# Autodesk Inventor assembly: belt drives
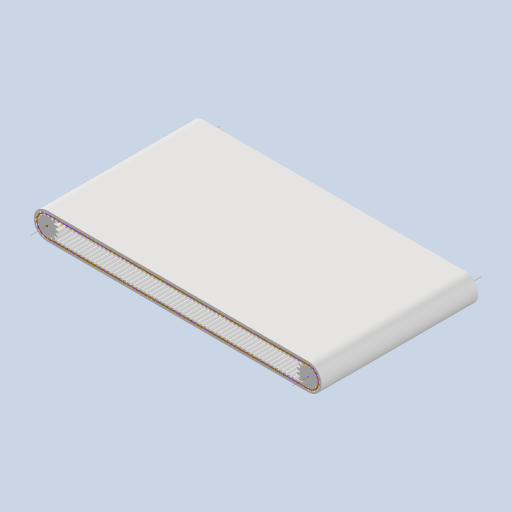
[picture p0: Inventor's stored thumbnail of the model, 512x512]
Saved by Autodesk Inventor 2024 (Build 280153000, 153)
## iProperties
Created: 2023-06-12
Part Number: belt drives
Document SubType Name: Assembly
Designer: ANIRUDH
Author: ANIRUDH
## Documents named in this file (5)
- C:\Users\ANIRUDH\Desktop\exploration\neha files\belt drives.iam
- C:\Users\ANIRUDH\Desktop\exploration\neha files\belt.ipt
- C:\Users\ANIRUDH\Desktop\exploration\neha files\gear-2.ipt
- C:\Users\ANIRUDH\Desktop\exploration\neha files\teeth-2.ipt
- C:\Users\ANIRUDH\Desktop\exploration\neha files\line3.ipt
## Components (135 placed, 4 different names)
1. belt:1 — Rigid:1, Rigid:2, Rotational:1, Rotational:2, Rotational:3, Rotational:4
2. gear-2:1 — Rotational:1
3. gear-2:2 — Rotational:2
4. line3:1 — Rotational:3
5. line3:2 — Rotational:4
6. teeth-2:1 — Rigid:1
7. teeth-2:2
8. teeth-2:3
9. teeth-2:4
10. teeth-2:5
11. teeth-2:6
12. teeth-2:7
13. teeth-2:8
14. teeth-2:9
15. teeth-2:10
16. teeth-2:11
17. teeth-2:12
18. teeth-2:13
19. teeth-2:14
20. teeth-2:15
21. teeth-2:16
22. teeth-2:17
23. teeth-2:18
24. teeth-2:19
25. teeth-2:20
26. teeth-2:21
27. teeth-2:22
28. teeth-2:23
29. teeth-2:24
30. teeth-2:25
31. teeth-2:26
32. teeth-2:27
33. teeth-2:28
34. teeth-2:29
35. teeth-2:30
36. teeth-2:31
37. teeth-2:32
38. teeth-2:33
39. teeth-2:34
40. teeth-2:35
41. teeth-2:36
42. teeth-2:37
43. teeth-2:38
44. teeth-2:39
45. teeth-2:40
46. teeth-2:41
47. teeth-2:42
48. teeth-2:43
49. teeth-2:44
50. teeth-2:45
51. teeth-2:46
52. teeth-2:47
53. teeth-2:48
54. teeth-2:49
55. teeth-2:50
56. teeth-2:51
57. teeth-2:52
58. teeth-2:53
59. teeth-2:54
60. teeth-2:55
61. teeth-2:56
62. teeth-2:57
63. teeth-2:58
64. teeth-2:59
65. teeth-2:60
66. teeth-2:61
67. teeth-2:62
68. teeth-2:63
69. teeth-2:64
70. teeth-2:65
71. teeth-2:66 — Rigid:2
72. teeth-2:67
73. teeth-2:68
74. teeth-2:69
75. teeth-2:70
76. teeth-2:71
77. teeth-2:72
78. teeth-2:73
79. teeth-2:74
80. teeth-2:75
81. teeth-2:76
82. teeth-2:77
83. teeth-2:78
84. teeth-2:79
85. teeth-2:80
86. teeth-2:81
87. teeth-2:82
88. teeth-2:83
89. teeth-2:84
90. teeth-2:85
91. teeth-2:86
92. teeth-2:87
93. teeth-2:88
94. teeth-2:89
95. teeth-2:90
96. teeth-2:91
97. teeth-2:92
98. teeth-2:93
99. teeth-2:94
100. teeth-2:95
101. teeth-2:96
102. teeth-2:97
103. teeth-2:98
104. teeth-2:99
105. teeth-2:100
106. teeth-2:101
107. teeth-2:102
108. teeth-2:103
109. teeth-2:104
110. teeth-2:105
111. teeth-2:106
112. teeth-2:107
113. teeth-2:108
114. teeth-2:109
115. teeth-2:110
116. teeth-2:111
117. teeth-2:112
118. teeth-2:113
119. teeth-2:114
120. teeth-2:115
121. teeth-2:116
122. teeth-2:117
123. teeth-2:118
124. teeth-2:119
125. teeth-2:120
126. teeth-2:121
127. teeth-2:122
128. teeth-2:123
129. teeth-2:124
130. teeth-2:125
131. teeth-2:126
132. teeth-2:127
133. teeth-2:128
134. teeth-2:129
135. teeth-2:130
## Component patterns: (65 elements, first: teeth-2:1), (65 elements, first: teeth-2:66)
## Relationships (6: RevoluteJoint 4, WeldJoint 2)
- Rigid:1 [WeldJoint]: belt:1 ↔ teeth-2:1
- Rigid:2 [WeldJoint]: belt:1 ↔ teeth-2:66
- Rotational:1 [RevoluteJoint]: belt:1 ↔ gear-2:1
- Rotational:2 [RevoluteJoint]: belt:1 ↔ gear-2:2
- Rotational:3 [RevoluteJoint]: belt:1 ↔ line3:1
- Rotational:4 [RevoluteJoint]: belt:1 ↔ line3:2
